# Autodesk Inventor assembly: Keyboard
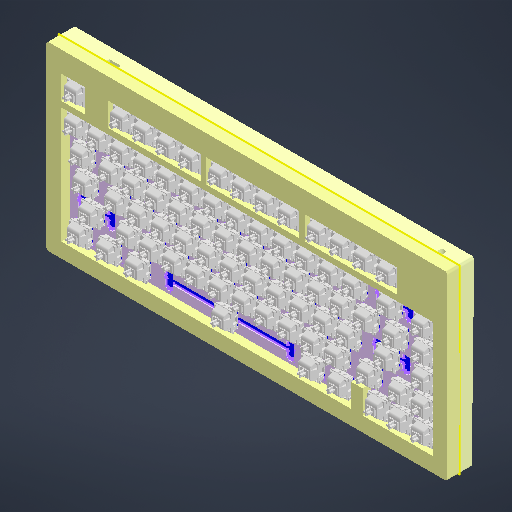
[picture p0: Inventor's stored thumbnail of the model, 512x512]
Saved by Autodesk Inventor 2026.1 (Build 301233000, 233)
## iProperties
Company: Kicad
Created: 2025-11-08
Part Number: Keyboard
Description: KiCad electronic assembly
Document SubType Name: Assembly
Designer: avani
Authority: Unknown
Sending System: KiCad to STEP converter
Preprocessor: Open CASCADE STEP processor 7.9
Title: Keyboard.step
Author: Pcbnew
## Documents named in this file (9)
- C:\Users\avani.DESKTOP-AVANISH\OneDrive\Documents\KiCad\Keyboard\Keyboard\Keyboard\Keyboard\Keyboard.iam
- C:\Users\avani.DESKTOP-AVANISH\OneDrive\Documents\KiCad\Keyboard\Keyboard\Keyboard\Keyboard\asm_mx_asm_PCB.iam
- C:\Users\avani.DESKTOP-AVANISH\OneDrive\Documents\KiCad\Keyboard\Keyboard\Keyboard\Keyboard\D_SOD-123.ipt
- C:\Users\avani.DESKTOP-AVANISH\OneDrive\Documents\KiCad\Keyboard\Keyboard\Keyboard\Keyboard\PJ-320.ipt
- C:\Users\avani.DESKTOP-AVANISH\OneDrive\Documents\KiCad\Keyboard\Keyboard\Keyboard\Keyboard\nice!nano v2.iam
- C:\Users\avani.DESKTOP-AVANISH\OneDrive\Documents\KiCad\Keyboard\Keyboard\Keyboard\Keyboard\Keyboard_PCB.ipt
- C:\Users\avani.DESKTOP-AVANISH\OneDrive\Documents\KiCad\Keyboard\Keyboard\Keyboard_Tray.ipt
- C:\Users\avani.DESKTOP-AVANISH\OneDrive\Documents\KiCad\Keyboard\Keyboard\Keyboard_Case.ipt
- C:\Users\avani.DESKTOP-AVANISH\OneDrive\Documents\KiCad\Keyboard\Keyboard\Keyboard_Plate.ipt
## Components (166 placed, 166 different names)
1. 7 [sub-assembly]
2. 8 [sub-assembly]
3. 9 [sub-assembly]
4. 10 [sub-assembly]
5. 11 [sub-assembly]
6. 12 [sub-assembly]
7. 13 [sub-assembly]
8. 14 [sub-assembly]
9. 15 [sub-assembly]
10. 16 [sub-assembly]
11. 17 [sub-assembly]
12. 18 [sub-assembly]
13. 19 [sub-assembly]
14. 20 [sub-assembly]
15. 21 [sub-assembly]
16. 22 [sub-assembly]
17. 23 [sub-assembly]
18. 24 [sub-assembly]
19. 25 [sub-assembly]
20. 26 [sub-assembly]
21. 27 [sub-assembly]
22. 28 [sub-assembly]
23. 29 [sub-assembly]
24. 30 [sub-assembly]
25. 31 [sub-assembly]
26. 32 [sub-assembly]
27. 33 [sub-assembly]
28. 34 [sub-assembly]
29. 35 [sub-assembly]
30. 36 [sub-assembly]
31. 37 [sub-assembly]
32. 38 [sub-assembly]
33. 39 [sub-assembly]
34. 40 [sub-assembly]
35. 41 [sub-assembly]
36. 42 [sub-assembly]
37. 43 [sub-assembly]
38. 44 [sub-assembly]
39. 45 [sub-assembly]
40. 46 [sub-assembly]
41. 47 [sub-assembly]
42. 48 [sub-assembly]
43. 49 [sub-assembly]
44. 50 [sub-assembly]
45. 51 [sub-assembly]
46. 52 [sub-assembly]
47. 53 [sub-assembly]
48. 54 [sub-assembly]
49. 55 [sub-assembly]
50. 56 [sub-assembly]
51. 57 [sub-assembly]
52. 58 [sub-assembly]
53. 59 [sub-assembly]
54. 60 [sub-assembly]
55. 61 [sub-assembly]
56. 62 [sub-assembly]
57. 63 [sub-assembly]
58. 64 [sub-assembly]
59. 65 [sub-assembly]
60. 66 [sub-assembly]
61. 67 [sub-assembly]
62. 68 [sub-assembly]
63. 69 [sub-assembly]
64. 70 [sub-assembly]
65. 71 [sub-assembly]
66. 72 [sub-assembly]
67. 73 [sub-assembly]
68. 74 [sub-assembly]
69. 75 [sub-assembly]
70. 76 [sub-assembly]
71. 77 [sub-assembly]
72. 78 [sub-assembly]
73. 79 [sub-assembly]
74. 80 [sub-assembly]
75. 81 [sub-assembly]
76. 82 [sub-assembly]
77. 83 [sub-assembly]
78. 84 [sub-assembly]
79. 85 [sub-assembly]
80. 86 [sub-assembly]
81. 87
82. 88
83. 89
84. 90
85. 91
86. 92
87. 93
88. 94
89. 95
90. 96
91. 97
92. 98
93. 99
94. 100
95. 101
96. 102
97. 103
98. 104
99. 105
100. 106
101. 107
102. 108
103. 109
104. 110
105. 111
106. 112
107. 113
108. 114
109. 115
110. 116
111. 117
112. 118
113. 119
114. 120
115. 121
116. 122
117. 123
118. 124
119. 125
120. 126
121. 127
122. 128
123. 129
124. 130
125. 131
126. 132
127. 133
128. 134
129. 135
130. 136
131. 137
132. 138
133. 139
134. 140
135. 141
136. 188 [sub-assembly]
137. 189
138. 190
139. 191
140. 192
141. 193
142. 194
143. 195
144. 196
145. 197
146. 198
147. 199
148. 200
149. 201
150. 202
151. 203
152. 204
153. 205
154. 206
155. 207
156. 208
157. 209
158. 210
159. 211
160. 212
161. 213
162. 214
163. 215 — Mate:1, Mate:2, Mate:3, Mate:4, Mate:7, Flush:7, Flush:8
164. Keyboard_Tray:1 — Mate:1, Mate:2, Mate:3, Mate:4, Mate:6, Flush:5, Flush:6
165. Keyboard_Case:1 — Mate:6, Flush:5, Flush:6
166. Keyboard_Plate:1 — Mate:7, Flush:7, Flush:8
## Relationships (10: Mate 6, Flush 4)
- Mate:1: 215 ↔ Keyboard_Tray:1
- Mate:2 (1.2025 mm): 215 ↔ Keyboard_Tray:1
- Mate:3 (1.2 mm): 215 ↔ Keyboard_Tray:1
- Mate:4: 215 ↔ Keyboard_Tray:1
- Mate:6: Keyboard_Tray:1 ↔ Keyboard_Case:1
- Flush:5: Keyboard_Tray:1 ↔ Keyboard_Case:1
- Flush:6: Keyboard_Tray:1 ↔ Keyboard_Case:1
- Mate:7: 215 ↔ Keyboard_Plate:1
- Flush:7: 215 ↔ Keyboard_Plate:1
- Flush:8: 215 ↔ Keyboard_Plate:1
